# Autodesk Inventor assembly: Structure
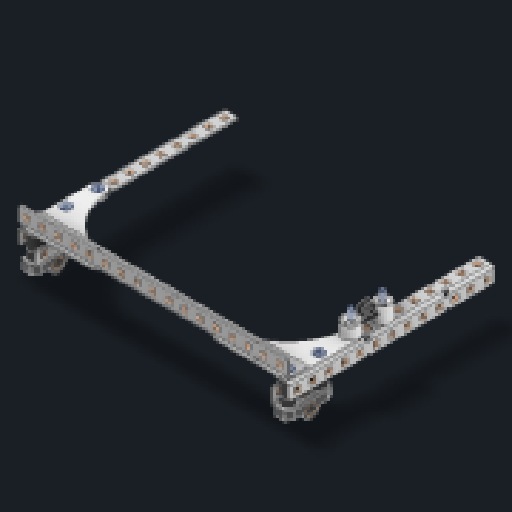
[picture p0: Inventor's stored thumbnail of the model, 512x512]
Saved by Autodesk Inventor 2025.1 (Build 291241000, 241)
## iProperties
Created: 2024-10-21
Part Number: Structure
Document SubType Name: Assembly
Designer: averey
Author: averey
## Documents named in this file (18)
- C:\Users\avere\VEX\High Stakes\CAD\V2\Intake\Floating Stage\Structure.iam
- C:\Users\avere\VEX\High Stakes\CAD\V2\Intake\Floating Stage\Left Angle Structure.iam
- C:\Users\avere\VEX\High Stakes\CAD\V2\Intake\Floating Stage\Right Angle Structure\Right Angle Structure.iam
- C:\Users\avere\VEX\High Stakes\CAD\ROBOPROS-CAD-Inventor\Structure\C Channel\Aluminum 1x3x1 Half Thick Cut\Alu C Half Thick 1x3x1x17.ipt
- C:\Users\avere\VEX\High Stakes\CAD\V2\Intake\Floating Stage\Custom Parts\Arm Triangle Gusset.ipt
- C:\Users\avere\VEX\High Stakes\CAD\ROBOPROS-CAD-Inventor\Structure\Hardware\Screw Shoulder Robosource\SScrew Shoulder Smooth .375 x .12.ipt
- C:\Users\avere\VEX\High Stakes\CAD\ROBOPROS-CAD-Inventor\Structure\Hardware\Screw Shoulder Robosource.ipt
- C:\Users\avere\VEX\High Stakes\CAD\ROBOPROS-CAD-Inventor\Structure\Hardware\Nut Nylon\Nut Nylon - White.ipt
- C:\Users\avere\VEX\High Stakes\CAD\ROBOPROS-CAD-Inventor\Structure\Hardware\Nut Nylon.ipt
- C:\Users\avere\VEX\High Stakes\CAD\ROBOPROS-CAD-Inventor\Structure\Hardware\Screw Steel - Star\SScrew Star Smooth 1.250.ipt
- C:\Users\avere\VEX\High Stakes\CAD\ROBOPROS-CAD-Inventor\Structure\Hardware\Screw Steel - Star.ipt
- C:\Users\avere\VEX\High Stakes\CAD\ROBOPROS-CAD-Inventor\Motion\Shaft LS\LS Pillow Bearing Block.ipt
- C:\Users\avere\VEX\High Stakes\CAD\ROBOPROS-CAD-Inventor\Motion\Spacers\Spacer Nylon .500 OD\NSpacer White .500 OD x .500.ipt
- C:\Users\avere\VEX\High Stakes\CAD\ROBOPROS-CAD-Inventor\Motion\Spacers\Spacer Nylon .500 OD.ipt
- C:\Users\avere\VEX\High Stakes\CAD\ROBOPROS-CAD-Inventor\Motion\Spacers\Spacer Nylon .500 OD\NSpacer White .500 OD x .375.ipt
- C:\Users\avere\VEX\High Stakes\CAD\ROBOPROS-CAD-Inventor\Motion\Spacers\Washer Steel\SWasher .500 OD x .062500\SWasher .500 OD x .062500.ipt
- C:\Users\avere\VEX\High Stakes\CAD\ROBOPROS-CAD-Inventor\Motion\Spacers\Washer Steel\SWasher .500 OD x .062500.ipt
- C:\Users\avere\VEX\High Stakes\CAD\ROBOPROS-CAD-Inventor\Structure\Hardware\Screw Steel - Star\SScrew Star Smooth .875.ipt
## Components (19 placed, 12 different names)
1. Left Angle Structure:1 [sub-assembly] — Mate:1, Mate:2, Flush:1, Mate:4, Insert:10, Insert:11, Insert:14, Insert:15
2. Right Angle Structure:1 [sub-assembly] — Flush:2, Mate:3, Flush:3, Insert:1
3. Alu C Half Thick 1x3x1x17:1 — Insert:1, Mate:4, Insert:2, Mate:5, Insert:3, Mate:6, Insert:6, Insert:7, Insert:8, Insert:9
4. Arm Triangle Gusset:1 — Insert:2, Mate:5, Insert:5
5. Arm Triangle Gusset:2 — Insert:3, Mate:6, Insert:4, Mate:7, Insert:12
6. SScrew Shoulder Smooth .375 x .12:1 — Insert:5
7. SScrew Shoulder Smooth .375 x .12:2 — Insert:4
8. Nut Nylon - White:1 — Insert:7
9. Nut Nylon - White:2 — Insert:6
10. SScrew Star Smooth 1.250:1 — Insert:8
11. SScrew Star Smooth 1.250:2 — Insert:9
12. LS Pillow Bearing Block:1 — Insert:10, Mate:7, Insert:16, Insert:17
13. NSpacer White .500 OD x .500:1 — Insert:11
14. NSpacer White .500 OD x .375:2 — Insert:12, Insert:13
15. SWasher .500 OD x .062500:1 — Insert:13
16. SScrew Star Smooth .875:3 — Insert:14
17. SScrew Star Smooth .875:4 — Insert:15
18. Nut Nylon - White:3 — Insert:17
19. Nut Nylon - White:4 — Insert:16
## Relationships (27: Insert 17, Mate 7, Flush 3)
- Mate:1 (96.4184 mm): Left Angle Structure:1
- Mate:2 (-82.55 mm): Left Angle Structure:1
- Flush:1: Left Angle Structure:1
- Flush:2: Right Angle Structure:1
- Mate:3 (-82.55 mm): Right Angle Structure:1
- Flush:3 (96.4184 mm): Right Angle Structure:1
- Insert:1 (1.5875 mm): Right Angle Structure:1 ↔ Alu C Half Thick 1x3x1x17:1
- Mate:4: Left Angle Structure:1 ↔ Alu C Half Thick 1x3x1x17:1
- Insert:2: Alu C Half Thick 1x3x1x17:1 ↔ Arm Triangle Gusset:1
- Mate:5: Alu C Half Thick 1x3x1x17:1 ↔ Arm Triangle Gusset:1
- Insert:3: Alu C Half Thick 1x3x1x17:1 ↔ Arm Triangle Gusset:2
- Mate:6: Alu C Half Thick 1x3x1x17:1 ↔ Arm Triangle Gusset:2
- Insert:4: Arm Triangle Gusset:2 ↔ SScrew Shoulder Smooth .375 x .12:2
- Insert:5: Arm Triangle Gusset:1 ↔ SScrew Shoulder Smooth .375 x .12:1
- Insert:6: Alu C Half Thick 1x3x1x17:1 ↔ Nut Nylon - White:2
- Insert:7: Alu C Half Thick 1x3x1x17:1 ↔ Nut Nylon - White:1
- Insert:8: Alu C Half Thick 1x3x1x17:1 ↔ SScrew Star Smooth 1.250:1
- Insert:9: Alu C Half Thick 1x3x1x17:1 ↔ SScrew Star Smooth 1.250:2
- Insert:10 (6.35 mm): Left Angle Structure:1 ↔ LS Pillow Bearing Block:1
- Mate:7: Arm Triangle Gusset:2 ↔ LS Pillow Bearing Block:1
- Insert:11: Left Angle Structure:1 ↔ NSpacer White .500 OD x .500:1
- Insert:12: Arm Triangle Gusset:2 ↔ NSpacer White .500 OD x .375:2
- Insert:13: NSpacer White .500 OD x .375:2 ↔ SWasher .500 OD x .062500:1
- Insert:14: Left Angle Structure:1 ↔ SScrew Star Smooth .875:3
- Insert:15: Left Angle Structure:1 ↔ SScrew Star Smooth .875:4
- Insert:16: LS Pillow Bearing Block:1 ↔ Nut Nylon - White:4
- Insert:17: LS Pillow Bearing Block:1 ↔ Nut Nylon - White:3
